# Autodesk Inventor assembly: Ensamble Extr
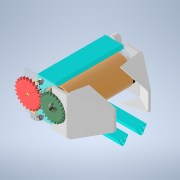
[picture p0: Inventor's stored thumbnail of the model, 180x180]
Saved by Autodesk Inventor 2020.3 (Build 243373000, 373)
## iProperties
Created: 2020-07-24
Part Number: Ensamble Extr
Document SubType Name: Assembly
Designer: juanp
Mass: 923.628 g
Surface Area: 3764.36 cm^2
Volume: 813.257 cm^3
Density: 1.13571 g/cm^3
Author: juanp
## Documents named in this file (16)
- C:\Users\juanp\Desktop\ROBOCOL\Idea Final NAF\Dispensador\Ensamble Dispensador.iam
- C:\Users\juanp\Desktop\ROBOCOL\Idea Final NAF\Dispensador\Tornillo.ipt
- C:\Users\juanp\Desktop\ROBOCOL\Idea Final NAF\Motor\DC Motor Gearbox.iam
- C:\Users\juanp\Desktop\ROBOCOL\Idea Final NAF\Dispensador\Eje.ipt
- C:\Users\juanp\Desktop\ROBOCOL\Idea Final NAF\Dispensador\Tubo Interior.ipt
- C:\Users\juanp\Desktop\ROBOCOL\Idea Final NAF\Dispensador\Tubo Exterior.ipt
- C:\Users\juanp\Desktop\ROBOCOL\Idea Final NAF\Dispensador\Engranaje B.ipt
- C:\Users\juanp\Desktop\ROBOCOL\Idea Final NAF\Dispensador\Engranaje A.ipt
- C:\Users\juanp\Documents\Inventor\Content Center Files\R2020\en-US\ANSI B18.16.3M(2)\ANSI B18.16.3M - Property Class 5 and 10 - Metric M5 x 0.8 Metal Type.ipt
- C:\Users\juanp\Desktop\ROBOCOL\Idea Final NAF\Dispensador\Tapa A.ipt
- C:\Users\juanp\Desktop\ROBOCOL\Idea Final NAF\Dispensador\Tapa B1.ipt
- C:\Users\juanp\Desktop\ROBOCOL\Idea Final NAF\Dispensador\Embudo.ipt
- C:\Users\juanp\Documents\Inventor\Content Center Files\R2020\en-US\JIS B 1174\JIS B 1174 - M5 x 25.ipt
- C:\Users\juanp\Desktop\ROBOCOL\Idea Final NAF\Dispensador\Adaptador.ipt
- C:\Users\juanp\Desktop\ROBOCOL\Idea Final NAF\Dispensador\Varilla M5.ipt
- C:\Users\juanp\Desktop\ROBOCOL\Idea Final NAF\Acoplador.ipt
## Components (23 placed, 15 different names)
1. Tornillo:1 — Mate:13, Flush:1, Angle:8
2. DC Motor Gearbox:1 [sub-assembly] — Flush:2, Mate:24, Mate:25, Mate:32, Flush:4
3. Eje:1 — Mate:13, Mate:15, Mate:33, Flush:8, Angle:9
4. Tubo Interior:1 — Mate:15, Mate:16, Mate:34, Tangent:1, Tangent:2
5. Tubo Exterior:1 — Mate:16, Flush:1, Flush:2, Mate:24, Mate:25, Mate:34, Mate:35, Mate:36, Mate:37, Mate:38, Mate:39, Mate:40, Mate:41, Mate:42, Angle:6, Angle:7, Mate:43, Mate:44, Flush:7
6. Prevailing Torque Type Hex Nut - Steel Metric Property Class 5 and 10 - Metric M5 x 0.8 Metal Type:1 — Mate:45, Mate:47
7. Prevailing Torque Type Hex Nut - Steel Metric Property Class 5 and 10 - Metric M5 x 0.8 Metal Type:2 — Mate:46, Mate:48
8. Engranaje B:1 — Mate:32, Flush:4, Flush:5, Angle:7
9. Engranaje A:1 — Mate:33, Flush:5, Angle:6, Angle:8, Angle:9
10. JIS B 1174 - Metric M5 x 25:1 — Mate:35, Tangent:1, Mate:46
11. JIS B 1174 - Metric M5 x 25:2 — Mate:36, Tangent:2, Mate:45
12. Tapa A:1 — Mate:37, Mate:38, Mate:39, Flush:8, Mate:49, Flush:9, Mate:50, Mate:53, Mate:54, Mate:63
13. Tapa B1:1 — Mate:40, Mate:41, Mate:42, Flush:10, Mate:51, Mate:52, Mate:59, Mate:60, Flush:11, Flush:12
14. Embudo:1 — Mate:43, Mate:44, Flush:7, Mate:47, Mate:48
15. Adaptador:1 — Flush:10, Mate:51, Mate:52
16. Adaptador:2 — Mate:49, Flush:9, Mate:50
17. Varilla M5:1 — Mate:53, Mate:56, Mate:61, Flush:11, Mate:64
18. Varilla M5:2 — Mate:54, Mate:55, Mate:62, Flush:12, Mate:65
19. Prevailing Torque Type Hex Nut - Steel Metric Property Class 5 and 10 - Metric M5 x 0.8 Metal Type:3 — Mate:56, Mate:66, Angle:10
20. Prevailing Torque Type Hex Nut - Steel Metric Property Class 5 and 10 - Metric M5 x 0.8 Metal Type:4 — Mate:55, Mate:67, Angle:11
21. Prevailing Torque Type Hex Nut - Steel Metric Property Class 5 and 10 - Metric M5 x 0.8 Metal Type:5 — Mate:60, Mate:62
22. Prevailing Torque Type Hex Nut - Steel Metric Property Class 5 and 10 - Metric M5 x 0.8 Metal Type:6 — Mate:59, Mate:61
23. Acoplador:1 — Mate:63, Mate:64, Mate:65, Mate:66, Mate:67, Angle:10, Angle:11
## Relationships (57: Mate 39, Flush 10, Angle 6, Tangent 2)
- Mate:13: Tornillo:1 ↔ Eje:1
- Mate:15: Eje:1 ↔ Tubo Interior:1
- Mate:16: Tubo Interior:1 ↔ Tubo Exterior:1
- Flush:1: Tornillo:1 ↔ Tubo Exterior:1
- Flush:2: DC Motor Gearbox:1 ↔ Tubo Exterior:1
- Mate:24: DC Motor Gearbox:1 ↔ Tubo Exterior:1
- Mate:25: DC Motor Gearbox:1 ↔ Tubo Exterior:1
- Mate:32: DC Motor Gearbox:1 ↔ Engranaje B:1
- Flush:4: DC Motor Gearbox:1 ↔ Engranaje B:1
- Mate:33: Eje:1 ↔ Engranaje A:1
- Flush:5: Engranaje B:1 ↔ Engranaje A:1
- Mate:34: Tubo Interior:1 ↔ Tubo Exterior:1
- Mate:35: Tubo Exterior:1 ↔ JIS B 1174 - Metric M5 x 25:1
- Mate:36: Tubo Exterior:1 ↔ JIS B 1174 - Metric M5 x 25:2
- Tangent:1: Tubo Interior:1 ↔ JIS B 1174 - Metric M5 x 25:1
- Tangent:2: Tubo Interior:1 ↔ JIS B 1174 - Metric M5 x 25:2
- Mate:37: Tubo Exterior:1 ↔ Tapa A:1
- Mate:38: Tubo Exterior:1 ↔ Tapa A:1
- Mate:39: Tubo Exterior:1 ↔ Tapa A:1
- Mate:40: Tubo Exterior:1 ↔ Tapa B1:1
- Mate:41: Tubo Exterior:1 ↔ Tapa B1:1
- Mate:42: Tubo Exterior:1 ↔ Tapa B1:1
- Angle:6 (760 deg): Tubo Exterior:1 ↔ Engranaje A:1
- Angle:7 (-760 deg): Tubo Exterior:1 ↔ Engranaje B:1
- Angle:8 (0 deg): Tornillo:1 ↔ Engranaje A:1
- Mate:43: Tubo Exterior:1 ↔ Embudo:1
- Mate:44: Tubo Exterior:1 ↔ Embudo:1
- Flush:7: Tubo Exterior:1 ↔ Embudo:1
- Mate:45: Prevailing Torque Type Hex Nut - Steel Metric Property Class 5 and 10 - Metric M5 x 0.8 Metal Type:1 ↔ JIS B 1174 - Metric M5 x 25:2
- Mate:46: Prevailing Torque Type Hex Nut - Steel Metric Property Class 5 and 10 - Metric M5 x 0.8 Metal Type:2 ↔ JIS B 1174 - Metric M5 x 25:1
- Mate:47: Prevailing Torque Type Hex Nut - Steel Metric Property Class 5 and 10 - Metric M5 x 0.8 Metal Type:1 ↔ Embudo:1
- Mate:48: Prevailing Torque Type Hex Nut - Steel Metric Property Class 5 and 10 - Metric M5 x 0.8 Metal Type:2 ↔ Embudo:1
- Flush:8: Eje:1 ↔ Tapa A:1
- Angle:9 (0 deg): Eje:1 ↔ Engranaje A:1
- Mate:49: Tapa A:1 ↔ Adaptador:2
- Flush:9: Tapa A:1 ↔ Adaptador:2
- Flush:10: Tapa B1:1 ↔ Adaptador:1
- Mate:50: Tapa A:1 ↔ Adaptador:2
- Mate:51: Tapa B1:1 ↔ Adaptador:1
- Mate:52: Tapa B1:1 ↔ Adaptador:1
- Mate:53: Tapa A:1 ↔ Varilla M5:1
- Mate:54: Tapa A:1 ↔ Varilla M5:2
- Mate:55: Varilla M5:2 ↔ Prevailing Torque Type Hex Nut - Steel Metric Property Class 5 and 10 - Metric M5 x 0.8 Metal Type:4
- Mate:56: Varilla M5:1 ↔ Prevailing Torque Type Hex Nut - Steel Metric Property Class 5 and 10 - Metric M5 x 0.8 Metal Type:3
- Mate:59: Tapa B1:1 ↔ Prevailing Torque Type Hex Nut - Steel Metric Property Class 5 and 10 - Metric M5 x 0.8 Metal Type:6
- Mate:60: Tapa B1:1 ↔ Prevailing Torque Type Hex Nut - Steel Metric Property Class 5 and 10 - Metric M5 x 0.8 Metal Type:5
- Mate:61: Varilla M5:1 ↔ Prevailing Torque Type Hex Nut - Steel Metric Property Class 5 and 10 - Metric M5 x 0.8 Metal Type:6
- Mate:62: Varilla M5:2 ↔ Prevailing Torque Type Hex Nut - Steel Metric Property Class 5 and 10 - Metric M5 x 0.8 Metal Type:5
- Flush:11 (-7 mm): Tapa B1:1 ↔ Varilla M5:1
- Flush:12 (-7 mm): Tapa B1:1 ↔ Varilla M5:2
- Mate:63: Tapa A:1 ↔ Acoplador:1
- Mate:64: Varilla M5:1 ↔ Acoplador:1
- Mate:65: Varilla M5:2 ↔ Acoplador:1
- Mate:66: Prevailing Torque Type Hex Nut - Steel Metric Property Class 5 and 10 - Metric M5 x 0.8 Metal Type:3 ↔ Acoplador:1
- Mate:67: Prevailing Torque Type Hex Nut - Steel Metric Property Class 5 and 10 - Metric M5 x 0.8 Metal Type:4 ↔ Acoplador:1
- Angle:10 (0 deg): Prevailing Torque Type Hex Nut - Steel Metric Property Class 5 and 10 - Metric M5 x 0.8 Metal Type:3 ↔ Acoplador:1
- Angle:11 (0 deg): Prevailing Torque Type Hex Nut - Steel Metric Property Class 5 and 10 - Metric M5 x 0.8 Metal Type:4 ↔ Acoplador:1
